# Autodesk Inventor assembly: Assem220
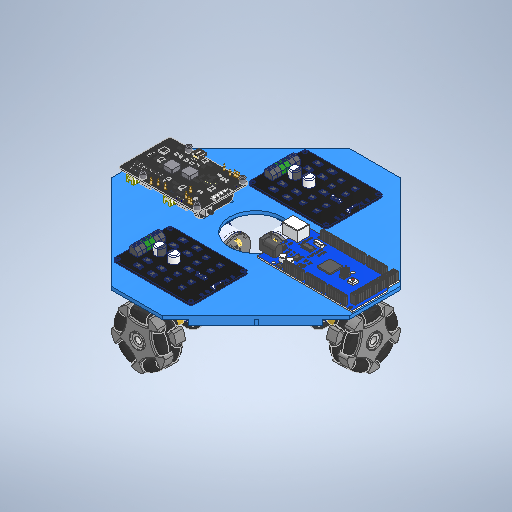
[picture p0: Inventor's stored thumbnail of the model, 512x512]
Saved by Autodesk Inventor 2025.1 (Build 291241000, 241)
## iProperties
Created: 2025-05-08
Part Number: Assem220
Document SubType Name: Assembly
Designer: User
Author: User
## Documents named in this file (12)
- D:\One Drive\OneDrive - Politeknik Sultan Salahuddin Abdul Aziz Shah\Documents\Inventor\RobosotPSA\Assem220.iam
- D:\One Drive\OneDrive - Politeknik Sultan Salahuddin Abdul Aziz Shah\Documents\Inventor\RobosotPSA\JGB37-520\JGB37-520\JGB37-520.ipt
- D:\One Drive\OneDrive - Politeknik Sultan Salahuddin Abdul Aziz Shah\Documents\Inventor\RobosotPSA\MM-JGB37 v4\MM-JGB37 v4\MM-JGB37 v4.ipt
- D:\One Drive\OneDrive - Politeknik Sultan Salahuddin Abdul Aziz Shah\Documents\Inventor\RobosotPSA\BASE.ipt
- D:\One Drive\OneDrive - Politeknik Sultan Salahuddin Abdul Aziz Shah\Documents\Inventor\RobosotPSA\geared motor brass coupling nut M12 nut 6mm shaft\geared motor brass coupling nut M12 nut 6mm shaft\geared moto.ipt
- D:\One Drive\OneDrive - Politeknik Sultan Salahuddin Abdul Aziz Shah\Documents\Inventor\RobosotPSA\omni_ext.ipt
- D:\One Drive\OneDrive - Politeknik Sultan Salahuddin Abdul Aziz Shah\Documents\Inventor\RobosotPSA\58mm Omni-Directional Wheel\58mm Omni-Directional Wheel\58mm Omni-Directional Wheel.ipt
- D:\One Drive\OneDrive - Politeknik Sultan Salahuddin Abdul Aziz Shah\Documents\Inventor\RobosotPSA\Template220.ipt
- D:\One Drive\OneDrive - Politeknik Sultan Salahuddin Abdul Aziz Shah\Documents\Inventor\RobosotPSA\MainBase.ipt
- D:\One Drive\OneDrive - Politeknik Sultan Salahuddin Abdul Aziz Shah\Documents\Inventor\RobosotPSA\Geekworm X1200 UPS HAT\Geekworm X1200 UPS HAT\Geekworm X1200 UPS HAT.ipt
- D:\One Drive\OneDrive - Politeknik Sultan Salahuddin Abdul Aziz Shah\Documents\Inventor\RobosotPSA\Arduino_Mega\Arduino_Mega\Arduino_Mega.ipt
- D:\One Drive\OneDrive - Politeknik Sultan Salahuddin Abdul Aziz Shah\Documents\Inventor\RobosotPSA\Motor Driver\Motor Driver\Motor Driver.ipt
## Components (30 placed, 11 different names)
1. Template220:1 — Flush:4
2. MainBase:1 — Flush:5, Mate:10, Mate:11, Mate:12, Mate:13
3. Geekworm X1200 UPS HAT:1 — Mate:10
4. Arduino_Mega:1 — Mate:11
5. Motor Driver:1 — Mate:12
6. Motor Driver:2 — Mate:13
7. JGB37-520:1 — Mate:2, Mate:3, Mate:4, Mate:5, Mate:6
8. MM-JGB37 v4:1 — Mate:1, Flush:1, Mate:2, Flush:2, Mate:3, Mate:4
9. BASE:1 — Mate:1, Flush:1, Flush:2, Flush:4
10. geared moto:1 — Mate:5, Mate:6, Flush:3, Mate:7
11. omni_ext:1 — Flush:3, Mate:7, Mate:8, Mate:9
12. 58mm Omni-Directional Wheel:1 — Mate:8, Mate:9
13. JGB37-520:3
14. MM-JGB37 v4:3
15. BASE:3
16. geared moto:3
17. omni_ext:3
18. 58mm Omni-Directional Wheel:3
19. JGB37-520:4
20. MM-JGB37 v4:4
21. BASE:4
22. geared moto:4
23. omni_ext:4
24. 58mm Omni-Directional Wheel:4
25. JGB37-520:5
26. MM-JGB37 v4:5 — Flush:5
27. BASE:5
28. geared moto:5
29. omni_ext:5
30. 58mm Omni-Directional Wheel:5
## Component patterns: (4 elements, first: JGB37-520:1 + MM-JGB37 v4:1 + BASE:1 + geared moto:1 + omni_ext:1 + 58mm Omni-Directional Wheel:1)
## Relationships (18: Mate 13, Flush 5)
- Mate:1: MM-JGB37 v4:1 ↔ BASE:1
- Flush:1: MM-JGB37 v4:1 ↔ BASE:1
- Mate:2: JGB37-520:1 ↔ MM-JGB37 v4:1
- Flush:2: MM-JGB37 v4:1 ↔ BASE:1
- Mate:3: JGB37-520:1 ↔ MM-JGB37 v4:1
- Mate:4: JGB37-520:1 ↔ MM-JGB37 v4:1
- Mate:5: JGB37-520:1 ↔ geared moto:1
- Mate:6: JGB37-520:1 ↔ geared moto:1
- Flush:3: geared moto:1 ↔ omni_ext:1
- Mate:7: geared moto:1 ↔ omni_ext:1
- Mate:8: omni_ext:1 ↔ 58mm Omni-Directional Wheel:1
- Mate:9: omni_ext:1 ↔ 58mm Omni-Directional Wheel:1
- Flush:4: Template220:1 ↔ BASE:1
- Flush:5: MainBase:1 ↔ MM-JGB37 v4:5
- Mate:10: MainBase:1 ↔ Geekworm X1200 UPS HAT:1
- Mate:11 (2 mm): MainBase:1 ↔ Arduino_Mega:1
- Mate:12 (2 mm): MainBase:1 ↔ Motor Driver:1
- Mate:13 (2 mm): MainBase:1 ↔ Motor Driver:2
